# Autodesk Inventor assembly: dormerScaffolding
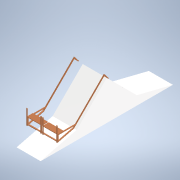
[picture p0: Inventor's stored thumbnail of the model, 180x180]
Saved by Autodesk Inventor 2021.1 (Build 251245000, 245)
## iProperties
Created: 2020-08-29
Part Number: dormerScaffolding
Document SubType Name: Assembly
Designer: robst
Author: robst
## Documents named in this file (4)
- C:\git\CAD-Development\robSteele\HouseProjects\dormerScaffolding\dormerScaffolding.iam
- C:\git\CAD-Development\robSteele\HouseProjects\dormerScaffolding\roof.ipt
- C:\git\CAD-Development\robSteele\HouseProjects\dormerScaffolding\side1.ipt
- C:\git\CAD-Development\robSteele\HouseProjects\dormerScaffolding\side1_MIR.ipt
## Components (3 placed, 3 different names)
1. roof:1 — Mate:1, Flush:1
2. side1:1 — Mate:1
3. side1_MIR:1
## Relationships (2: Mate 1, Flush 1)
- Mate:1: roof:1 ↔ side1:1
- Flush:1 (-1828.8 mm): roof:1
